# Autodesk Inventor assembly: Assembly3
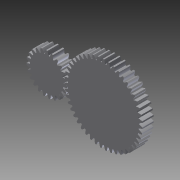
[picture p0: Inventor's stored thumbnail of the model, 180x180]
Saved by Autodesk Inventor 2012 (Build 160160000, 160)
## iProperties
Created: 2013-11-18
Part Number: Assembly3
Document SubType Name: Assembly
Designer: fqian3
Author: fqian3
## Documents named in this file (4)
- D:\Jessica\Inventor\Assembly3.iam
- D:\Dropbox\Research\Heterogeneous\Kugel\3Dprint\Part5.ipt
- D:\Dropbox\Research\Heterogeneous\Kugel\3Dprint\Part6.ipt
- D:\Dropbox\Research\Heterogeneous\Kugel\3Dprint\Assembly3\Design Accelerator\Spur Gears1.iam
## Components (3 placed, 3 different names)
1. Part5:1 — Flush:1
2. Spur Gears:1 [sub-assembly]
3. Part6:1 — Flush:1
## Relationships (1: Flush 1)
- Flush:1: Part5:1 ↔ Part6:1
